# Autodesk Inventor assembly: enc-BackPanel MitteLinks - Assembly
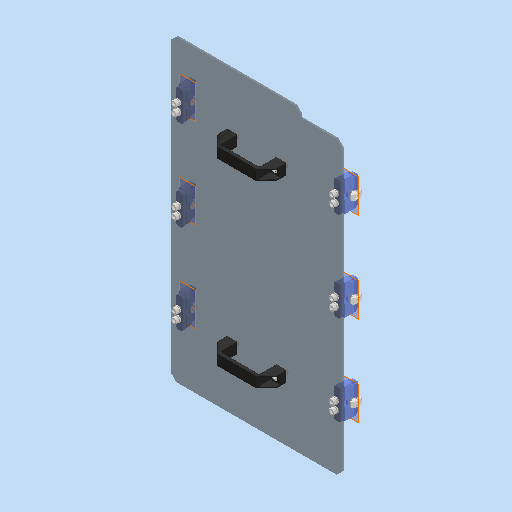
[picture p0: Inventor's stored thumbnail of the model, 512x512]
Saved by Autodesk Inventor 2023.2 (Build 272271000, 271)
## iProperties
Created: 2023-12-04
Part Number: enc-BackPanel MitteLinks - Assembly
Document SubType Name: Assembly
Designer: Nils Bade
Author: Nils Bade
## Documents named in this file (6)
- C:\Users\nilsb\Documents\Inventor\Projektarbeit-Bade\Enclosure\enc-BackPanel MitteLinks - Assembly.iam
- C:\Users\nilsb\Documents\Inventor\Projektarbeit-Bade\Enclosure\V-Slot Door Handle v1.ipt
- C:\Users\nilsb\Documents\Inventor\Projektarbeit-Bade\Schrauben\Cap Head Screw M6x16 - DIN912.ipt
- C:\Users\nilsb\Documents\Inventor\Projektarbeit-Bade\RatRig_Standards\Hex Locking Nut - M6 v2.ipt
- C:\Users\nilsb\Documents\Inventor\Projektarbeit-Bade\Enclosure\Magnet PanelFrame 90deg connected.iam
- C:\Users\nilsb\Documents\Inventor\Projektarbeit-Bade\Enclosure\enc-BackPanel Mitte.ipt
## Components (17 placed, 5 different names)
1. enc-BackPanel Mitte:1
2. V-Slot Door Handle v1:1 — Passend:12, Passend:13, Passend:21, Passend:22
3. V-Slot Door Handle v1:2 — Passend:17, Passend:18, Passend:19, Passend:20
4. Cap Head Screw M6x16 - DIN912:1 — Passend:3, Passend:12, Passend:22
5. Cap Head Screw M6x16 - DIN912:2 — Passend:4, Passend:13, Passend:21
6. Cap Head Screw M6x16 - DIN912:3 — Passend:2, Passend:18, Passend:19
7. Cap Head Screw M6x16 - DIN912:4 — Passend:1, Passend:17, Passend:20
8. Hex Locking Nut - M6 v2:1 — Passend:3
9. Hex Locking Nut - M6 v2:2 — Passend:4
10. Hex Locking Nut - M6 v2:3 — Passend:2
11. Hex Locking Nut - M6 v2:4 — Passend:1
12. Magnet PanelFrame 90deg connected:1 [sub-assembly]
13. Magnet PanelFrame 90deg connected:2 [sub-assembly]
14. Magnet PanelFrame 90deg connected:3 [sub-assembly]
15. Magnet PanelFrame 90deg connected:4 [sub-assembly]
16. Magnet PanelFrame 90deg connected:5 [sub-assembly]
17. Magnet PanelFrame 90deg connected:6 [sub-assembly]
## Relationships (40: Mate 40)
- Passend:1 [Mate]: Cap Head Screw M6x16 - DIN912:4 ↔ Hex Locking Nut - M6 v2:4
- Passend:2 [Mate]: Cap Head Screw M6x16 - DIN912:3 ↔ Hex Locking Nut - M6 v2:3
- Passend:3 [Mate]: Cap Head Screw M6x16 - DIN912:1 ↔ Hex Locking Nut - M6 v2:1
- Passend:4 [Mate]: Cap Head Screw M6x16 - DIN912:2 ↔ Hex Locking Nut - M6 v2:2
- [Mate]: enc-BackPanel Mitte:1 ↔ Hex Locking Nut - M6 v2:1
- [Mate]: enc-BackPanel Mitte:1 ↔ Hex Locking Nut - M6 v2:2
- [Mate]: enc-BackPanel Mitte:1 ↔ Hex Locking Nut - M6 v2:4
- [Mate]: enc-BackPanel Mitte:1 ↔ Hex Locking Nut - M6 v2:3
- [Mate]: enc-BackPanel Mitte:1 ↔ V-Slot Door Handle v1:1
- [Mate]: enc-BackPanel Mitte:1 ↔ V-Slot Door Handle v1:1
- [Mate]: enc-BackPanel Mitte:1 ↔ V-Slot Door Handle v1:1
- Passend:12 [Mate]: V-Slot Door Handle v1:1 ↔ Cap Head Screw M6x16 - DIN912:1
- Passend:13 [Mate]: V-Slot Door Handle v1:1 ↔ Cap Head Screw M6x16 - DIN912:2
- [Mate]: enc-BackPanel Mitte:1 ↔ V-Slot Door Handle v1:2
- [Mate]: enc-BackPanel Mitte:1 ↔ V-Slot Door Handle v1:2
- [Mate]: enc-BackPanel Mitte:1 ↔ V-Slot Door Handle v1:2
- Passend:17 [Mate]: V-Slot Door Handle v1:2 ↔ Cap Head Screw M6x16 - DIN912:4
- Passend:18 [Mate]: V-Slot Door Handle v1:2 ↔ Cap Head Screw M6x16 - DIN912:3
- Passend:19 [Mate]: V-Slot Door Handle v1:2 ↔ Cap Head Screw M6x16 - DIN912:3
- Passend:20 [Mate]: V-Slot Door Handle v1:2 ↔ Cap Head Screw M6x16 - DIN912:4
- Passend:21 [Mate]: V-Slot Door Handle v1:1 ↔ Cap Head Screw M6x16 - DIN912:2
- Passend:22 [Mate]: V-Slot Door Handle v1:1 ↔ Cap Head Screw M6x16 - DIN912:1
- [Mate]: enc-BackPanel Mitte:1 ↔ Magnet PanelFrame 90deg connected:4
- [Mate]: enc-BackPanel Mitte:1 ↔ Magnet PanelFrame 90deg connected:4
- [Mate]: enc-BackPanel Mitte:1 ↔ Magnet PanelFrame 90deg connected:4
- [Mate]: enc-BackPanel Mitte:1 ↔ Magnet PanelFrame 90deg connected:5
- [Mate]: enc-BackPanel Mitte:1 ↔ Magnet PanelFrame 90deg connected:5
- [Mate]: enc-BackPanel Mitte:1 ↔ Magnet PanelFrame 90deg connected:5
- [Mate]: enc-BackPanel Mitte:1 ↔ Magnet PanelFrame 90deg connected:6
- [Mate]: enc-BackPanel Mitte:1 ↔ Magnet PanelFrame 90deg connected:6
- [Mate]: enc-BackPanel Mitte:1 ↔ Magnet PanelFrame 90deg connected:6
- [Mate]: enc-BackPanel Mitte:1 ↔ Magnet PanelFrame 90deg connected:1
- [Mate]: enc-BackPanel Mitte:1 ↔ Magnet PanelFrame 90deg connected:1
- [Mate]: enc-BackPanel Mitte:1 ↔ Magnet PanelFrame 90deg connected:1
- [Mate]: enc-BackPanel Mitte:1 ↔ Magnet PanelFrame 90deg connected:2
- [Mate]: enc-BackPanel Mitte:1 ↔ Magnet PanelFrame 90deg connected:2
- [Mate]: enc-BackPanel Mitte:1 ↔ Magnet PanelFrame 90deg connected:2
- [Mate]: enc-BackPanel Mitte:1 ↔ Magnet PanelFrame 90deg connected:3
- [Mate]: enc-BackPanel Mitte:1 ↔ Magnet PanelFrame 90deg connected:3
- [Mate]: enc-BackPanel Mitte:1 ↔ Magnet PanelFrame 90deg connected:3
